# Autodesk Inventor assembly: Ellbow n24_v2
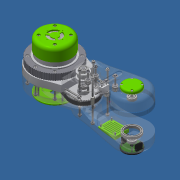
[picture p0: Inventor's stored thumbnail of the model, 180x180]
Saved by Autodesk Inventor 2016 (Build 200138000, 138)
## iProperties
Created: 2015-08-24
Part Number: Ellbow n24_v2
Material: Generisch
Document SubType Name: Assembly
Designer: 4ndreas
Mass: 4086.83 g
Surface Area: 5319.91 cm^2
Volume: 2356.13 cm^3
Density: 1.73455 g/cm^3
Author: 4ndreas
## Documents named in this file (42)
- C:\Users\4ndreas\Documents\Inventor\RobotARM v2\v4\_assemblys\Elbow.iam
- C:\Users\4ndreas\Documents\Inventor\RobotARM v2\v4\Elbow\Konstruktions-Assistent\Übertragung des Zahnriemens1.iam
- C:\Users\4ndreas\Documents\Inventor\RobotARM v2\v4\_motors\Nema24.ipt
- C:\Users\4ndreas\Documents\Inventor\RobotARM v2\v4\Elbow\Konstruktions-Assistent\Übertragung des Zahnriemens2.iam
- C:\Users\4ndreas\Documents\Inventor\RobotARM v2\v4\_printed parts\OberArm_A.ipt
- C:\Users\4ndreas\Documents\Inventor\RobotARM v2\v4\_printed parts\OberArm_B.ipt
- C:\Users\4ndreas\Documents\Inventor\RobotARM v2\v4\_misc parts\OberArm_C.ipt
- C:\Users\4ndreas\Documents\Inventor\RobotARM v2\v4\Elbow\Konstruktions-Assistent\Welle1.iam
- C:\Users\4ndreas\Documents\Inventor\Content Center Files\R2014\de-DE\DIN BEARING(1)\DIN 625 SKF - SKF 608.ipt
- C:\Users\4ndreas\Documents\Inventor\RobotARM v2\v4\_assemblys\encoder.iam
- C:\Users\4ndreas\Documents\Inventor\RobotARM v2\v4\_standard Parts\DIN 912 - M4 x 0,7 x50.ipt
- C:\Users\4ndreas\Documents\Inventor\RobotARM v2\v4\_printed parts\MotorCoverN24_3.ipt
- C:\Users\4ndreas\Documents\Inventor\RobotARM v2\v4\_printed parts\Cover_G2.ipt
- C:\Users\4ndreas\Documents\Inventor\Content Center Files\R2014\de-DE\DIN 912\DIN 912 - M3 x 0,5 x 10 x 8,75.ipt
- C:\Users\4ndreas\Documents\Inventor\Content Center Files\R2014\de-DE\DIN 912\DIN 912 - M4 x 0,7 x 35 x 20.ipt
- C:\Users\4ndreas\Documents\Inventor\Content Center Files\R2014\de-DE\DIN 912\DIN 912 - M4 x 0,7 x 40 x 20.ipt
- C:\Users\4ndreas\Documents\Inventor\Content Center Files\R2014\de-DE\DIN 9021\DIN 9021 - 4,3.ipt
- C:\Users\4ndreas\Documents\Inventor\Content Center Files\R2014\de-DE\DIN 625 - T1\DIN 625 T1 - 624 - 4 x 13 x 5.ipt
- C:\Users\4ndreas\Documents\Inventor\Content Center Files\R2014\de-DE\DIN 125-1  A\DIN 125 - A 4,3.ipt
- C:\Users\4ndreas\Documents\Inventor\Content Center Files\R2014\de-DE\DIN BEARING(1)\DIN 625 SKF - SKF 61807.ipt
- C:\Users\4ndreas\Documents\Inventor\RobotARM v2\v4\_standard Parts\DIN 912 - M4 x 0,7 x55.ipt
- C:\Users\4ndreas\Documents\Inventor\RobotARM v2\v4\_metal parts\16221600.ipt
- C:\Users\4ndreas\Documents\Inventor\Content Center Files\R2014\de-DE\DIN 912\DIN 912 - M4 x 0,7 x 30 x 20.ipt
- C:\Users\4ndreas\Documents\Inventor\Content Center Files\R2014\de-DE\DIN 933\DIN 933 - M4  x 55.ipt
- C:\Users\4ndreas\Documents\Inventor\Content Center Files\R2014\de-DE\DIN 934\DIN 934 - M4 x 0,7.ipt
- C:\Users\4ndreas\Documents\Inventor\Content Center Files\R2014\de-DE\DIN 562\DIN 562 - M4 x 7.ipt
- C:\Users\4ndreas\Documents\Inventor\Content Center Files\R2014\de-DE\DIN 933\DIN 933 - M4  x 25.ipt
- C:\Users\4ndreas\Documents\Inventor\RobotARM v2\v4\_printed parts\OberArmMagnet.ipt
- C:\Users\4ndreas\Documents\Inventor\Content Center Files\R2014\de-DE\DIN 7991(2)\DIN 7991 - M4x30.ipt
- C:\Users\4ndreas\Documents\Inventor\RobotARM v2\v4\_metal parts\Synchrone RiemenscheibeT5_z48.ipt
- C:\Users\4ndreas\Documents\Inventor\RobotARM v2\v4\_metal parts\Belt_T_Spacer.ipt
- C:\Users\4ndreas\Documents\Inventor\RobotARM v2\v4\_standard Parts\DIN 625 SKF - SKF 624_flansch.ipt
- C:\Users\4ndreas\Documents\Inventor\Content Center Files\R2014\de-DE\DIN 125-1  A\DIN 125 - A 8,4.ipt
- C:\Users\4ndreas\Documents\Inventor\Content Center Files\R2014\de-DE\DIN 933\DIN 933 - M4  x 40.ipt
- C:\Users\4ndreas\Documents\Inventor\RobotARM v2\v4\_encoder\EncoderMagnet.ipt
- C:\Users\4ndreas\Documents\Inventor\RobotARM v2\v4\_printed parts\Cable_Cover.ipt
- C:\Users\4ndreas\Documents\Inventor\RobotARM v2\v4\_metal parts\Alu_Belt_tens.ipt
- C:\Users\4ndreas\Documents\Inventor\Content Center Files\R2014\de-DE\DIN 913\DIN 913 - M4 x 16.ipt
- C:\Users\4ndreas\Documents\Inventor\RobotARM v2\v4\_standard Parts\Distanzhuelse_M4x20mm.ipt
- C:\Users\4ndreas\Documents\Inventor\Content Center Files\R2014\de-DE\DIN 913\DIN 913 - M4 x 4.ipt
- C:\Users\4ndreas\Documents\Inventor\Content Center Files\R2014\de-DE\BS EN ISO 13337\ISO 13337 - 3 x 26BS EN ISO.ipt
- C:\Users\4ndreas\Documents\Inventor\Content Center Files\R2014\de-DE\BS EN ISO 13337\ISO 13337 - 3 x 20BS EN ISO.ipt
## Components (175 placed, 40 different names)
1. Übertragung des Zahnriemens:1 [sub-assembly] — Passend:25, Passend:31, Passend:37, Passend:41, Passend:120, Passend:193
2. Nema24:1 — Passend:3, Passend:16, Winkel:1, Winkel:2, Passend:33, Passend:35, Passend:36, Passend:52, Passend:54, Passend:55, Passend:154, Passend:155, Fluchtend:11
3. Übertragung des Zahnriemens:2 [sub-assembly] — Passend:16, Passend:24, Passend:34, Passend:156
4. OberArm_A:1 — Passend:29, Fluchtend:1, Passend:30, Fluchtend:3, Passend:32, Passend:33, Passend:34, Passend:44, Passend:45, Passend:72, Passend:73, Passend:74, Passend:75, Passend:76, Passend:78, Passend:245, Passend:246, Passend:247, Passend:248, Passend:249, Passend:275, Passend:283, Winkel:3, Passend:291, Passend:292
5. OberArm_B:1 — Passend:28, Passend:29, Fluchtend:1, Passend:30, Fluchtend:4, Passend:43, Passend:50, Passend:226, Passend:227, Passend:228, Passend:229, Passend:241, Passend:242, Passend:243, Passend:244, Fluchtend:12, Passend:273
6. OberArm_C:1 — Passend:28, Fluchtend:3, Passend:31, Fluchtend:4, Passend:48, Passend:49, Passend:51, Fluchtend:9, Passend:102, Passend:103, Passend:107, Passend:108, Passend:130, Passend:131, Passend:132, Passend:133, Passend:134, Passend:135, Passend:136, Passend:137, Passend:138, Passend:144, Passend:150, Passend:151, Passend:161, Passend:162, Passend:201, Passend:202, Passend:203, Passend:204, Passend:205, Passend:211, Passend:220, Passend:222, Passend:223, Passend:250, Passend:251, Passend:252, Passend:256, Fluchtend:17, Passend:319, Passend:320, Passend:105, Passend:324, Passend:325, Passend:336, Passend:339, Passend:340
7. Cover_G2:1 — Fluchtend:9, Passend:80, Passend:81, Passend:82, Passend:83, Passend:84, Passend:85, Passend:86, Passend:87
8. Welle:1 [sub-assembly] — Passend:37, Passend:38, Passend:40, Passend:39, Passend:206, Passend:284, Passend:286, Passend:287, Tangential:1
9. encoder:1 [sub-assembly] — Passend:41, Passend:43, Passend:256
10. OberArmMagnet:1 — Fluchtend:12, Passend:261, Passend:262, Fluchtend:13, Passend:263, Passend:264, Fluchtend:14, Fluchtend:15, Passend:310, Passend:311
11. DIN 625 SKF SKF 608:1 — Passend:38, Passend:204
12. DIN 625 SKF SKF 608:2 — Passend:39, Passend:205, Passend:207
13. DIN 625 SKF SKF 608:3 — Passend:40, Passend:203
14. DIN 625 SKF SKF 608:4 — Passend:45, Passend:49
15. DIN 625 SKF SKF 608:5 — Passend:50, Passend:51
16. DIN 625 SKF SKF 608:6 — Passend:44, Passend:48
17. DIN 912 - ersetzt durch DIN EN ISO 4762 M4 x 50:5 — Passend:55, Passend:71, Passend:258
18. DIN 912 - ersetzt durch DIN EN ISO 4762 M4 x 50:6 — Passend:54, Passend:69
19. DIN 912 - ersetzt durch DIN EN ISO 4762 M4 x 50:7 — Passend:53, Passend:70
20. DIN 912 - ersetzt durch DIN EN ISO 4762 M4 x 50:8 — Passend:52, Passend:68
21. DIN 125-1 A A 4,3:6
22. DIN 125-1 A A 4,3:7
23. DIN 125-1 A A 4,3:8
24. DIN 125-1 A A 4,3:9
25. Distanzhuelse_M4x20mm:1 — Passend:71, Fluchtend:6, Fluchtend:7, Passend:72
26. Distanzhuelse_M4x20mm:2 — Passend:69, Fluchtend:6, Passend:73, Passend:88
27. Distanzhuelse_M4x20mm:3 — Passend:70, Fluchtend:7, Fluchtend:8, Passend:75, Passend:76
28. Distanzhuelse_M4x20mm:4 — Passend:68, Fluchtend:8, Passend:74, Passend:259
29. MotorCoverN24_3:1 — Passend:78, Passend:89, Passend:92, Passend:93, Passend:94, Passend:257, Passend:260
30. DIN 912 - ersetzt durch DIN EN ISO 4762 M3 x 10:1 — Passend:82, Passend:87
31. DIN 912 - ersetzt durch DIN EN ISO 4762 M3 x 10:2 — Passend:81, Passend:86
32. DIN 912 - ersetzt durch DIN EN ISO 4762 M3 x 10:3 — Passend:83, Passend:84
33. DIN 912 - ersetzt durch DIN EN ISO 4762 M3 x 10:4 — Passend:80, Passend:85
34. DIN 912 - ersetzt durch DIN EN ISO 4762 M4 x 35:1 — Passend:88, Passend:89
35. DIN 912 - ersetzt durch DIN EN ISO 4762 M4 x 35:2 — Passend:92, Passend:93, Passend:258
36. DIN 912 - ersetzt durch DIN EN ISO 4762 M4 x 35:3 — Passend:259, Passend:260
37. DIN 912 - ersetzt durch DIN EN ISO 4762 M4 x 35:4 — Passend:90, Passend:94, Passend:257
38. DIN 933 - ersetzt durch DIN EN 24017 M4  x 40:1 — Passend:96, Passend:105, Passend:109, Passend:115, Passend:121, Passend:293, Passend:296, Passend:297
39. DIN 9021 4,3:1 — Passend:96, Passend:102, Passend:298
40. DIN 9021 4,3:2 — Passend:103, Passend:303, Passend:307, Fluchtend:18
41. DIN 9021 4,3:3 — Passend:108, Passend:109, Passend:122
42. DIN 9021 4,3:4 — Passend:107, Passend:123, Passend:309, Passend:323
43. DIN 625 - T1 624 - 4 x 13 x 5:1 — Passend:110, Passend:124, Passend:294
44. F624 ZZ 4x13x5:2 — Passend:110, Passend:115, Passend:295, Passend:296
45. DIN 625 - T1 624 - 4 x 13 x 5:3 — Passend:125, Passend:304, Passend:305
46. DIN 125-1 A A 4,3:1 — Passend:117, Passend:119, Passend:125, Passend:308
47. DIN 125-1 A A 4,3:2 — Passend:117, Passend:119, Passend:120, Passend:123
48. DIN 125-1 A A 4,3:3 — Passend:116, Passend:118, Passend:124
49. DIN 125-1 A A 4,3:4 — Passend:116, Passend:118, Passend:121, Passend:122
50. DIN 625 SKF SKF 61807:1 — Passend:130, Passend:131
51. Distanzhuelse_M4x20mm:5 — Passend:132, Passend:136, Passend:137
52. Distanzhuelse_M4x20mm:6 — Passend:133, Passend:134, Passend:135
53. DIN 912 - ersetzt durch DIN EN ISO 4762 M4 x 55:12 — Passend:138
54. DIN 125-1 A A 4,3:10
55. DIN 912 - ersetzt durch DIN EN ISO 4762 M4 x 55:13 — Passend:144
56. DIN 125-1 A A 4,3:11
57. DIN 912 - ersetzt durch DIN EN ISO 4762 M4 x 55:14 — Passend:151
58. DIN 125-1 A A 4,3:12
59. DIN 912 - ersetzt durch DIN EN ISO 4762 M4 x 55:15 — Passend:150
60. DIN 125-1 A A 4,3:13
61. 16221600:1 — Passend:154, Passend:155, Fluchtend:10, Passend:345
62. Synchrone RiemenscheibeT5_z48:1 — Passend:156, Fluchtend:10, Passend:285, Passend:289, Passend:341, Passend:342
63. DIN 912 - ersetzt durch DIN EN ISO 4762 M4 x 55:16 — Passend:162, Passend:190
64. DIN 912 - ersetzt durch DIN EN ISO 4762 M4 x 55:17 — Passend:161, Passend:165, Passend:188
65. DIN 125-1 A A 4,3:14
66. DIN 125-1 A A 4,3:15
67. DIN 912 - ersetzt durch DIN EN ISO 4762 M4 x 30:1 — Passend:165, Passend:187
68. DIN 125-1 A A 4,3:16
69. DIN 125-1 A A 4,3:17
70. DIN 933 - ersetzt durch DIN EN 24017 M4  x 55:2 — Passend:184, Passend:191, Passend:192, Passend:198
71. DIN 933 - ersetzt durch DIN EN 24017 M4  x 55:1 — Passend:183, Passend:194, Passend:196
72. DIN 125-1 A A 4,3:18
73. DIN 125-1 A A 4,3:19
74. DIN 934 - ersetzt durch DIN EN 24032/28673/28674 M4:1 — Passend:188
75. DIN 934 - ersetzt durch DIN EN 24032/28673/28674 M4:2 — Passend:187
76. DIN 934 - ersetzt durch DIN EN 24032/28673/28674 M4:3 — Passend:184
77. DIN 934 - ersetzt durch DIN EN 24032/28673/28674 M4:4 — Passend:183
78. DIN 934 - ersetzt durch DIN EN 24032/28673/28674 M4:6 — Passend:190
79. DIN 625 - T1 624 - 4 x 13 x 5:5 — Passend:193, Passend:195, Passend:197
80. DIN 625 - T1 624 - 4 x 13 x 5:6 — Passend:192, Passend:199, Passend:201
81. DIN 625 - T1 624 - 4 x 13 x 5:7 — Passend:191, Passend:199, Passend:200
82. DIN 625 - T1 624 - 4 x 13 x 5:8 — Passend:194, Passend:195, Passend:202
83. DIN 934 - ersetzt durch DIN EN 24032/28673/28674 M4:7 — Passend:196, Passend:197
84. DIN 934 - ersetzt durch DIN EN 24032/28673/28674 M4:8 — Passend:198, Passend:200
85. 16221600:2 — Passend:206, Passend:207, Passend:288, Passend:343, Passend:344
86. DIN 912 - ersetzt durch DIN EN ISO 4762 M4 x 55:18 — Passend:211, Passend:239
87. DIN 125-1 A A 4,3:20
88. DIN 912 - ersetzt durch DIN EN ISO 4762 M4 x 55:19 — Passend:220, Passend:240
89. DIN 912 - ersetzt durch DIN EN ISO 4762 M4 x 55:20 — Passend:222, Passend:238
90. DIN 912 - ersetzt durch DIN EN ISO 4762 M4 x 55:21 — Passend:223, Passend:237
91. DIN 125-1 A A 4,3:21
92. DIN 125-1 A A 4,3:5
93. DIN 125-1 A A 4,3:22
94. DIN 562 M4:1 — Passend:239, Passend:245, Passend:246
95. DIN 562 M4:2 — Passend:240, Passend:241, Passend:242
96. DIN 562 M4:3 — Passend:237, Passend:247, Passend:248
97. DIN 562 M4:4 — Passend:238, Passend:243, Passend:244
98. DIN 933 - ersetzt durch DIN EN 24017 M4  x 25:1 — Passend:250, Passend:251, Passend:252, Passend:254
99. DIN 934 - ersetzt durch DIN EN 24032/28673/28674 M4:9 — Passend:254
100. DIN 7991 M4x30:2 — Passend:262, Fluchtend:13, Passend:267
101. DIN 7991 M4x30:3 — Passend:263, Fluchtend:14, Passend:266
102. DIN 7991 M4x30:4 — Passend:264, Fluchtend:15, Passend:269
103. DIN 7991 M4x30:1 — Passend:268
104. DIN 934 - ersetzt durch DIN EN 24032/28673/28674 M4:10 — Passend:268, Passend:272
105. DIN 934 - ersetzt durch DIN EN 24032/28673/28674 M4:11 — Passend:267, Passend:271, Passend:272, Passend:273
106. DIN 934 - ersetzt durch DIN EN 24032/28673/28674 M4:12 — Passend:269, Passend:270
107. DIN 934 - ersetzt durch DIN EN 24032/28673/28674 M4:13 — Passend:266, Passend:270, Passend:271
108. Belt_T_Spacer:1 — Passend:274, Passend:275, Passend:281, Winkel:3
109. DIN 912 - ersetzt durch DIN EN ISO 4762 M4 x 40:11 — Passend:274, Passend:276, Passend:277, Passend:278, Passend:282, Passend:283, Passend:290
110. F624 ZZ 4x13x5:1 — Passend:276, Passend:280, Passend:281
111. DIN 625 - T1 624 - 4 x 13 x 5:9 — Passend:278, Passend:279, Passend:282
112. DIN 125-1 A A 4,3:37 — Passend:277, Passend:279, Passend:280
113. DIN 125-1 A A 8,4:1 — Passend:284, Passend:285
114. DIN 125-1 A A 8,4:2 — Passend:287, Passend:288
115. DIN 125-1 A A 8,4:3 — Passend:286, Passend:289
116. DIN 562 M4:5 — Passend:290, Passend:291, Passend:292
117. DIN 125-1 A A 4,3:38 — Passend:293, Passend:294, Passend:295
118. DIN 934 - ersetzt durch DIN EN 24032/28673/28674 M4:14 — Passend:297, Passend:298
119. F624 ZZ 4x13x5:3 — Passend:299, Passend:300, Passend:302
120. DIN 933 - ersetzt durch DIN EN 24017 M4  x 40:2 — Passend:299, Passend:300, Passend:301, Passend:303, Passend:305, Passend:306, Passend:308, Passend:309, Passend:322
121. DIN 934 - ersetzt durch DIN EN 24032/28673/28674 M4:15 — Passend:306, Passend:307
122. DIN 125-1 A A 4,3:39 — Passend:301, Passend:302, Passend:304
123. EncoderMagnet:1 — Passend:310, Passend:311
124. Cable_Cover:1 — Fluchtend:17, Passend:312, Passend:313, Passend:314, Passend:315, Passend:316, Passend:317, Passend:318, Passend:321
125. DIN 912 - ersetzt durch DIN EN ISO 4762 M3 x 10:5 — Passend:314, Passend:316
126. DIN 912 - ersetzt durch DIN EN ISO 4762 M3 x 10:6 — Passend:315, Passend:319, Passend:321
127. DIN 912 - ersetzt durch DIN EN ISO 4762 M3 x 10:7 — Passend:313, Passend:317
128. DIN 912 - ersetzt durch DIN EN ISO 4762 M3 x 10:8 — Passend:312, Passend:318, Passend:320
129. Alu_Belt_tens:1 — Passend:322, Passend:323, Passend:328, Passend:332, Passend:338
130. DIN 912 - ersetzt durch DIN EN ISO 4762 M4 x 30:18 — Passend:328, Passend:329, Passend:330, Passend:331, Passend:333, Passend:335
131. DIN 9021 4,3:5 — Passend:329, Fluchtend:18, Passend:330
132. DIN 9021 4,3:7 — Passend:331, Passend:332, Passend:334
133. DIN 934 - ersetzt durch DIN EN 24032/28673/28674 M4:16 — Passend:333, Passend:334
134. DIN 934 - ersetzt durch DIN EN 24032/28673/28674 M4:17 — Passend:336, Passend:337, Passend:339, Passend:340
135. DIN 913 M4 x 16:1 — Passend:337, Passend:338
136. DIN 913 M4 x 4:1 — Passend:341, Tangential:1
137. BS EN ISO 13337 3 x 26:1 — Passend:342
138. DIN 913 M4 x 4:2 — Passend:343
139. BS EN ISO 13337 3 x 20:1 — Passend:344
140. DIN 913 M4 x 4:3 — Passend:345
141. DIN 912 - ersetzt durch DIN EN ISO 4762 M4 x 30:5 — Passend:229
142. DIN 125-1 A A 4,3:23
143. Distanzhuelse_M4x20mm:7 — Passend:226, Passend:227, Passend:228, Passend:235
144. DIN 912 - ersetzt durch DIN EN ISO 4762 M4 x 30:4 — Passend:235
145. DIN 125-1 A A 4,3:24
146. DIN 912 - ersetzt durch DIN EN ISO 4762 M4 x 30:6
147. DIN 125-1 A A 4,3:25
148. Distanzhuelse_M4x20mm:8
149. DIN 912 - ersetzt durch DIN EN ISO 4762 M4 x 30:7
150. DIN 125-1 A A 4,3:26
151. DIN 912 - ersetzt durch DIN EN ISO 4762 M4 x 30:8
152. DIN 125-1 A A 4,3:27
153. Distanzhuelse_M4x20mm:9
154. DIN 912 - ersetzt durch DIN EN ISO 4762 M4 x 30:9
155. DIN 125-1 A A 4,3:28
156. DIN 912 - ersetzt durch DIN EN ISO 4762 M4 x 30:10
157. DIN 125-1 A A 4,3:29
158. Distanzhuelse_M4x20mm:10
159. DIN 912 - ersetzt durch DIN EN ISO 4762 M4 x 30:11
160. DIN 125-1 A A 4,3:30
161. DIN 912 - ersetzt durch DIN EN ISO 4762 M4 x 30:12
162. DIN 125-1 A A 4,3:31
163. Distanzhuelse_M4x20mm:11
164. DIN 912 - ersetzt durch DIN EN ISO 4762 M4 x 30:13
165. DIN 125-1 A A 4,3:32
166. DIN 912 - ersetzt durch DIN EN ISO 4762 M4 x 30:14
167. DIN 125-1 A A 4,3:33
168. Distanzhuelse_M4x20mm:12
169. DIN 912 - ersetzt durch DIN EN ISO 4762 M4 x 30:15
170. DIN 125-1 A A 4,3:34
171. DIN 912 - ersetzt durch DIN EN ISO 4762 M4 x 30:16
172. DIN 125-1 A A 4,3:35
173. Distanzhuelse_M4x20mm:13
174. DIN 912 - ersetzt durch DIN EN ISO 4762 M4 x 30:17
175. DIN 125-1 A A 4,3:36
## Component patterns: (7 elements, first: DIN 912 - ersetzt durch DIN EN ISO 4762 M4 x 30:5 + DIN 125-1 A A 4,3:23 + Distanzhuelse_M4x20mm:7 + DIN 912 - ersetzt durch DIN EN ISO 4762 M4 x 30:4 + DIN 125-1 A A 4,3:24)
## Relationships (316: Mate 296, Flush 16, Angle 3, Tangent 1)
- Passend:3 [Mate]: Nema24:1
- Passend:12 [Mate]
- Passend:13 [Mate]
- Passend:16 [Mate]: Nema24:1 ↔ Übertragung des Zahnriemens:2
- Winkel:1 [Angle] (0 deg): Nema24:1
- Passend:24 [Mate]: Übertragung des Zahnriemens:2
- Passend:25 [Mate]: Übertragung des Zahnriemens:1
- Winkel:2 [Angle] (180 deg): Nema24:1
- Passend:28 [Mate]: OberArm_B:1 ↔ OberArm_C:1
- Passend:29 [Mate]: OberArm_A:1 ↔ OberArm_B:1
- Fluchtend:1 [Flush]: OberArm_A:1 ↔ OberArm_B:1
- Passend:30 [Mate]: OberArm_A:1 ↔ OberArm_B:1
- Fluchtend:3 [Flush]: OberArm_A:1 ↔ OberArm_C:1
- Passend:31 [Mate]: Übertragung des Zahnriemens:1 ↔ OberArm_C:1
- Passend:32 [Mate]: OberArm_A:1
- Passend:33 [Mate]: Nema24:1 ↔ OberArm_A:1
- Passend:34 [Mate]: Übertragung des Zahnriemens:2 ↔ OberArm_A:1
- Passend:35 [Mate]: Nema24:1
- Passend:36 [Mate]: Nema24:1
- Fluchtend:4 [Flush]: OberArm_B:1 ↔ OberArm_C:1
- Passend:37 [Mate]: Übertragung des Zahnriemens:1 ↔ Welle:1
- Passend:38 [Mate]: Welle:1 ↔ DIN 625 SKF SKF 608:1
- Passend:39 [Mate]: Welle:1 ↔ DIN 625 SKF SKF 608:2
- Passend:40 [Mate]: Welle:1 ↔ DIN 625 SKF SKF 608:3
- Passend:41 [Mate]: Übertragung des Zahnriemens:1 ↔ encoder:1
- Passend:43 [Mate]: OberArm_B:1 ↔ encoder:1
- Passend:44 [Mate]: OberArm_A:1 ↔ DIN 625 SKF SKF 608:6
- Passend:45 [Mate]: OberArm_A:1 ↔ DIN 625 SKF SKF 608:4
- Passend:48 [Mate]: OberArm_C:1 ↔ DIN 625 SKF SKF 608:6
- Passend:49 [Mate]: OberArm_C:1 ↔ DIN 625 SKF SKF 608:4
- Passend:50 [Mate]: OberArm_B:1 ↔ DIN 625 SKF SKF 608:5
- Passend:51 [Mate]: OberArm_C:1 ↔ DIN 625 SKF SKF 608:5
- Passend:52 [Mate]: Nema24:1 ↔ DIN 912 - ersetzt durch DIN EN ISO 4762 M4 x 50:8
- Passend:53 [Mate]: DIN 912 - ersetzt durch DIN EN ISO 4762 M4 x 50:7
- Passend:54 [Mate]: Nema24:1 ↔ DIN 912 - ersetzt durch DIN EN ISO 4762 M4 x 50:6
- Passend:55 [Mate]: Nema24:1 ↔ DIN 912 - ersetzt durch DIN EN ISO 4762 M4 x 50:5
- [Mate]: DIN 912 - ersetzt durch DIN EN ISO 4762 M4 x 50:8 ↔ DIN 125-1 A A 4,3:7
- [Mate]: DIN 912 - ersetzt durch DIN EN ISO 4762 M4 x 50:6 ↔ DIN 125-1 A A 4,3:6
- [Mate]: DIN 912 - ersetzt durch DIN EN ISO 4762 M4 x 50:5 ↔ DIN 125-1 A A 4,3:9
- [Mate]: DIN 912 - ersetzt durch DIN EN ISO 4762 M4 x 50:7 ↔ DIN 125-1 A A 4,3:8
- [Mate]: DIN 912 - ersetzt durch DIN EN ISO 4762 M4 x 50:7 ↔ DIN 125-1 A A 4,3:8
- [Mate]: DIN 912 - ersetzt durch DIN EN ISO 4762 M4 x 50:8 ↔ DIN 125-1 A A 4,3:7
- [Mate]: DIN 912 - ersetzt durch DIN EN ISO 4762 M4 x 50:6 ↔ DIN 125-1 A A 4,3:6
- [Mate]: DIN 912 - ersetzt durch DIN EN ISO 4762 M4 x 50:5 ↔ DIN 125-1 A A 4,3:9
- [Mate]: Nema24:1 ↔ DIN 125-1 A A 4,3:6
- [Mate]: Nema24:1 ↔ DIN 125-1 A A 4,3:7
- [Mate]: Nema24:1 ↔ DIN 125-1 A A 4,3:9
- [Mate]: Nema24:1 ↔ DIN 125-1 A A 4,3:8
- Passend:68 [Mate]: DIN 912 - ersetzt durch DIN EN ISO 4762 M4 x 50:8 ↔ Distanzhuelse_M4x20mm:4
- Passend:69 [Mate]: DIN 912 - ersetzt durch DIN EN ISO 4762 M4 x 50:6 ↔ Distanzhuelse_M4x20mm:2
- Passend:70 [Mate]: DIN 912 - ersetzt durch DIN EN ISO 4762 M4 x 50:7 ↔ Distanzhuelse_M4x20mm:3
- Passend:71 [Mate]: DIN 912 - ersetzt durch DIN EN ISO 4762 M4 x 50:5 ↔ Distanzhuelse_M4x20mm:1
- Fluchtend:6 [Flush]: Distanzhuelse_M4x20mm:1 ↔ Distanzhuelse_M4x20mm:2
- Fluchtend:7 [Flush]: Distanzhuelse_M4x20mm:1 ↔ Distanzhuelse_M4x20mm:3
- Fluchtend:8 [Flush]: Distanzhuelse_M4x20mm:3 ↔ Distanzhuelse_M4x20mm:4
- Passend:72 [Mate]: OberArm_A:1 ↔ Distanzhuelse_M4x20mm:1
- Passend:73 [Mate]: OberArm_A:1 ↔ Distanzhuelse_M4x20mm:2
- Passend:74 [Mate]: OberArm_A:1 ↔ Distanzhuelse_M4x20mm:4
- Passend:75 [Mate]: OberArm_A:1 ↔ Distanzhuelse_M4x20mm:3
- Passend:76 [Mate]: OberArm_A:1 ↔ Distanzhuelse_M4x20mm:3
- Passend:78 [Mate]: OberArm_A:1 ↔ MotorCoverN24_3:1
- Fluchtend:9 [Flush]: OberArm_C:1 ↔ Cover_G2:1
- Passend:80 [Mate]: Cover_G2:1 ↔ DIN 912 - ersetzt durch DIN EN ISO 4762 M3 x 10:4
- Passend:81 [Mate]: Cover_G2:1 ↔ DIN 912 - ersetzt durch DIN EN ISO 4762 M3 x 10:2
- Passend:82 [Mate]: Cover_G2:1 ↔ DIN 912 - ersetzt durch DIN EN ISO 4762 M3 x 10:1
- Passend:83 [Mate]: Cover_G2:1 ↔ DIN 912 - ersetzt durch DIN EN ISO 4762 M3 x 10:3
- Passend:84 [Mate]: Cover_G2:1 ↔ DIN 912 - ersetzt durch DIN EN ISO 4762 M3 x 10:3
- Passend:85 [Mate]: Cover_G2:1 ↔ DIN 912 - ersetzt durch DIN EN ISO 4762 M3 x 10:4
- Passend:86 [Mate]: Cover_G2:1 ↔ DIN 912 - ersetzt durch DIN EN ISO 4762 M3 x 10:2
- Passend:87 [Mate]: Cover_G2:1 ↔ DIN 912 - ersetzt durch DIN EN ISO 4762 M3 x 10:1
- Passend:88 [Mate]: Distanzhuelse_M4x20mm:2 ↔ DIN 912 - ersetzt durch DIN EN ISO 4762 M4 x 35:1
- Passend:89 [Mate]: MotorCoverN24_3:1 ↔ DIN 912 - ersetzt durch DIN EN ISO 4762 M4 x 35:1
- Passend:90 [Mate]: DIN 912 - ersetzt durch DIN EN ISO 4762 M4 x 35:4
- Passend:92 [Mate]: MotorCoverN24_3:1 ↔ DIN 912 - ersetzt durch DIN EN ISO 4762 M4 x 35:2
- Passend:93 [Mate]: MotorCoverN24_3:1 ↔ DIN 912 - ersetzt durch DIN EN ISO 4762 M4 x 35:2
- Passend:94 [Mate]: MotorCoverN24_3:1 ↔ DIN 912 - ersetzt durch DIN EN ISO 4762 M4 x 35:4
- Passend:96 [Mate]: DIN 933 - ersetzt durch DIN EN 24017 M4  x 40:1 ↔ DIN 9021 4,3:1
- Passend:102 [Mate]: OberArm_C:1 ↔ DIN 9021 4,3:1
- Passend:103 [Mate]: OberArm_C:1 ↔ DIN 9021 4,3:2
- Passend:105 [Mate]: OberArm_C:1 ↔ DIN 933 - ersetzt durch DIN EN 24017 M4  x 40:1
- Passend:107 [Mate]: OberArm_C:1 ↔ DIN 9021 4,3:4
- Passend:108 [Mate]: OberArm_C:1 ↔ DIN 9021 4,3:3
- Passend:109 [Mate]: DIN 933 - ersetzt durch DIN EN 24017 M4  x 40:1 ↔ DIN 9021 4,3:3
- Passend:110 [Mate]: DIN 625 - T1 624 - 4 x 13 x 5:1 ↔ F624 ZZ 4x13x5:2
- Passend:115 [Mate]: DIN 933 - ersetzt durch DIN EN 24017 M4  x 40:1 ↔ F624 ZZ 4x13x5:2
- Passend:116 [Mate]: DIN 125-1 A A 4,3:3 ↔ DIN 125-1 A A 4,3:4
- Passend:117 [Mate]: DIN 125-1 A A 4,3:1 ↔ DIN 125-1 A A 4,3:2
- Passend:118 [Mate]: DIN 125-1 A A 4,3:3 ↔ DIN 125-1 A A 4,3:4
- Passend:119 [Mate]: DIN 125-1 A A 4,3:1 ↔ DIN 125-1 A A 4,3:2
- Passend:120 [Mate]: Übertragung des Zahnriemens:1 ↔ DIN 125-1 A A 4,3:2
- Passend:121 [Mate]: DIN 933 - ersetzt durch DIN EN 24017 M4  x 40:1 ↔ DIN 125-1 A A 4,3:4
- Passend:122 [Mate]: DIN 9021 4,3:3 ↔ DIN 125-1 A A 4,3:4
- Passend:123 [Mate]: DIN 9021 4,3:4 ↔ DIN 125-1 A A 4,3:2
- Passend:124 [Mate]: DIN 625 - T1 624 - 4 x 13 x 5:1 ↔ DIN 125-1 A A 4,3:3
- Passend:125 [Mate]: DIN 625 - T1 624 - 4 x 13 x 5:3 ↔ DIN 125-1 A A 4,3:1
- Passend:130 [Mate]: OberArm_C:1 ↔ DIN 625 SKF SKF 61807:1
- Passend:131 [Mate]: OberArm_C:1 ↔ DIN 625 SKF SKF 61807:1
- Passend:132 [Mate]: OberArm_C:1 ↔ Distanzhuelse_M4x20mm:5
- Passend:133 [Mate]: OberArm_C:1 ↔ Distanzhuelse_M4x20mm:6
- Passend:134 [Mate]: OberArm_C:1 ↔ Distanzhuelse_M4x20mm:6
- Passend:135 [Mate]: OberArm_C:1 ↔ Distanzhuelse_M4x20mm:6
- Passend:136 [Mate]: OberArm_C:1 ↔ Distanzhuelse_M4x20mm:5
- Passend:137 [Mate]: OberArm_C:1 ↔ Distanzhuelse_M4x20mm:5
- Passend:138 [Mate]: OberArm_C:1 ↔ DIN 912 - ersetzt durch DIN EN ISO 4762 M4 x 55:12
- [Mate]: DIN 912 - ersetzt durch DIN EN ISO 4762 M4 x 55:12 ↔ DIN 125-1 A A 4,3:10
- [Mate]: DIN 912 - ersetzt durch DIN EN ISO 4762 M4 x 55:12 ↔ DIN 125-1 A A 4,3:10
- [Mate]: OberArm_C:1 ↔ DIN 125-1 A A 4,3:10
- [Mate]: DIN 912 - ersetzt durch DIN EN ISO 4762 M4 x 55:13 ↔ DIN 125-1 A A 4,3:11
- [Mate]: DIN 912 - ersetzt durch DIN EN ISO 4762 M4 x 55:13 ↔ DIN 125-1 A A 4,3:11
- Passend:144 [Mate]: OberArm_C:1 ↔ DIN 912 - ersetzt durch DIN EN ISO 4762 M4 x 55:13
- [Mate]: OberArm_C:1 ↔ DIN 125-1 A A 4,3:11
- [Mate]: DIN 912 - ersetzt durch DIN EN ISO 4762 M4 x 55:14 ↔ DIN 125-1 A A 4,3:12
- [Mate]: DIN 912 - ersetzt durch DIN EN ISO 4762 M4 x 55:14 ↔ DIN 125-1 A A 4,3:12
- [Mate]: DIN 912 - ersetzt durch DIN EN ISO 4762 M4 x 55:15 ↔ DIN 125-1 A A 4,3:13
- [Mate]: DIN 912 - ersetzt durch DIN EN ISO 4762 M4 x 55:15 ↔ DIN 125-1 A A 4,3:13
- Passend:150 [Mate]: OberArm_C:1 ↔ DIN 912 - ersetzt durch DIN EN ISO 4762 M4 x 55:15
- Passend:151 [Mate]: OberArm_C:1 ↔ DIN 912 - ersetzt durch DIN EN ISO 4762 M4 x 55:14
- [Mate]: OberArm_C:1 ↔ DIN 125-1 A A 4,3:12
- [Mate]: OberArm_C:1 ↔ DIN 125-1 A A 4,3:13
- Passend:154 [Mate]: Nema24:1 ↔ 16221600:1
- Passend:155 [Mate] (1 mm): Nema24:1 ↔ 16221600:1
- Passend:156 [Mate]: Übertragung des Zahnriemens:2 ↔ Synchrone RiemenscheibeT5_z48:1
- Fluchtend:10 [Flush]: 16221600:1 ↔ Synchrone RiemenscheibeT5_z48:1
- Fluchtend:11 [Flush] (7 mm): Nema24:1
- [Mate]: DIN 912 - ersetzt durch DIN EN ISO 4762 M4 x 55:17 ↔ DIN 125-1 A A 4,3:15
- [Mate]: DIN 912 - ersetzt durch DIN EN ISO 4762 M4 x 55:16 ↔ DIN 125-1 A A 4,3:14
- [Mate]: DIN 912 - ersetzt durch DIN EN ISO 4762 M4 x 55:16 ↔ DIN 125-1 A A 4,3:14
- [Mate]: DIN 912 - ersetzt durch DIN EN ISO 4762 M4 x 55:17 ↔ DIN 125-1 A A 4,3:15
- Passend:161 [Mate]: OberArm_C:1 ↔ DIN 912 - ersetzt durch DIN EN ISO 4762 M4 x 55:17
- Passend:162 [Mate]: OberArm_C:1 ↔ DIN 912 - ersetzt durch DIN EN ISO 4762 M4 x 55:16
- [Mate]: OberArm_C:1 ↔ DIN 125-1 A A 4,3:14
- [Mate]: OberArm_C:1 ↔ DIN 125-1 A A 4,3:15
- Passend:165 [Mate]: DIN 912 - ersetzt durch DIN EN ISO 4762 M4 x 55:17 ↔ DIN 912 - ersetzt durch DIN EN ISO 4762 M4 x 30:1
- [Mate]: DIN 912 - ersetzt durch DIN EN ISO 4762 M4 x 30:1 ↔ DIN 125-1 A A 4,3:17
- [Mate]: DIN 912 - ersetzt durch DIN EN ISO 4762 M4 x 30:1 ↔ DIN 125-1 A A 4,3:17
- [Mate]: OberArm_C:1 ↔ DIN 125-1 A A 4,3:16
- [Mate]: OberArm_C:1 ↔ DIN 125-1 A A 4,3:17
- [Mate]: Übertragung des Zahnriemens:1 ↔ DIN 933 - ersetzt durch DIN EN 24017 M4  x 55:2
- [Mate]: Übertragung des Zahnriemens:1 ↔ DIN 933 - ersetzt durch DIN EN 24017 M4  x 55:1
- [Mate]: OberArm_C:1 ↔ DIN 933 - ersetzt durch DIN EN 24017 M4  x 55:2
- [Mate]: OberArm_C:1 ↔ DIN 933 - ersetzt durch DIN EN 24017 M4  x 55:1
- [Mate]: OberArm_C:1 ↔ DIN 933 - ersetzt durch DIN EN 24017 M4  x 55:2
- [Mate]: OberArm_C:1 ↔ DIN 933 - ersetzt durch DIN EN 24017 M4  x 55:1
- [Mate]: OberArm_C:1 ↔ DIN 125-1 A A 4,3:18
- [Mate]: OberArm_C:1 ↔ DIN 125-1 A A 4,3:19
- [Mate]: DIN 933 - ersetzt durch DIN EN 24017 M4  x 55:2 ↔ DIN 125-1 A A 4,3:19
- [Mate]: DIN 933 - ersetzt durch DIN EN 24017 M4  x 55:1 ↔ DIN 125-1 A A 4,3:18
- Passend:183 [Mate]: DIN 933 - ersetzt durch DIN EN 24017 M4  x 55:1 ↔ DIN 934 - ersetzt durch DIN EN 24032/28673/28674 M4:4
- Passend:184 [Mate]: DIN 933 - ersetzt durch DIN EN 24017 M4  x 55:2 ↔ DIN 934 - ersetzt durch DIN EN 24032/28673/28674 M4:3
- [Mate]: DIN 125-1 A A 4,3:19 ↔ DIN 934 - ersetzt durch DIN EN 24032/28673/28674 M4:3
- [Mate]: DIN 125-1 A A 4,3:18 ↔ DIN 934 - ersetzt durch DIN EN 24032/28673/28674 M4:4
- Passend:187 [Mate]: DIN 912 - ersetzt durch DIN EN ISO 4762 M4 x 30:1 ↔ DIN 934 - ersetzt durch DIN EN 24032/28673/28674 M4:2
- Passend:188 [Mate]: DIN 912 - ersetzt durch DIN EN ISO 4762 M4 x 55:17 ↔ DIN 934 - ersetzt durch DIN EN 24032/28673/28674 M4:1
- Passend:190 [Mate]: DIN 912 - ersetzt durch DIN EN ISO 4762 M4 x 55:16 ↔ DIN 934 - ersetzt durch DIN EN 24032/28673/28674 M4:6
- Passend:191 [Mate]: DIN 933 - ersetzt durch DIN EN 24017 M4  x 55:2 ↔ DIN 625 - T1 624 - 4 x 13 x 5:7
- Passend:192 [Mate]: DIN 933 - ersetzt durch DIN EN 24017 M4  x 55:2 ↔ DIN 625 - T1 624 - 4 x 13 x 5:6
- Passend:193 [Mate]: Übertragung des Zahnriemens:1 ↔ DIN 625 - T1 624 - 4 x 13 x 5:5
- Passend:194 [Mate]: DIN 933 - ersetzt durch DIN EN 24017 M4  x 55:1 ↔ DIN 625 - T1 624 - 4 x 13 x 5:8
- Passend:195 [Mate]: DIN 625 - T1 624 - 4 x 13 x 5:5 ↔ DIN 625 - T1 624 - 4 x 13 x 5:8
- Passend:196 [Mate]: DIN 933 - ersetzt durch DIN EN 24017 M4  x 55:1 ↔ DIN 934 - ersetzt durch DIN EN 24032/28673/28674 M4:7
- Passend:197 [Mate]: DIN 625 - T1 624 - 4 x 13 x 5:5 ↔ DIN 934 - ersetzt durch DIN EN 24032/28673/28674 M4:7
- Passend:198 [Mate]: DIN 933 - ersetzt durch DIN EN 24017 M4  x 55:2 ↔ DIN 934 - ersetzt durch DIN EN 24032/28673/28674 M4:8
- Passend:199 [Mate]: DIN 625 - T1 624 - 4 x 13 x 5:6 ↔ DIN 625 - T1 624 - 4 x 13 x 5:7
- Passend:200 [Mate]: DIN 625 - T1 624 - 4 x 13 x 5:7 ↔ DIN 934 - ersetzt durch DIN EN 24032/28673/28674 M4:8
- Passend:201 [Mate]: OberArm_C:1 ↔ DIN 625 - T1 624 - 4 x 13 x 5:6
- Passend:202 [Mate]: OberArm_C:1 ↔ DIN 625 - T1 624 - 4 x 13 x 5:8
- Passend:203 [Mate]: OberArm_C:1 ↔ DIN 625 SKF SKF 608:3
- Passend:204 [Mate]: OberArm_C:1 ↔ DIN 625 SKF SKF 608:1
- Passend:205 [Mate]: OberArm_C:1 ↔ DIN 625 SKF SKF 608:2
- Passend:206 [Mate]: Welle:1 ↔ 16221600:2
- Passend:207 [Mate] (0.5 mm): DIN 625 SKF SKF 608:2 ↔ 16221600:2
- [Mate]: DIN 912 - ersetzt durch DIN EN ISO 4762 M4 x 55:18 ↔ DIN 125-1 A A 4,3:20
- [Mate]: DIN 912 - ersetzt durch DIN EN ISO 4762 M4 x 55:18 ↔ DIN 125-1 A A 4,3:20
- [Mate]: OberArm_C:1 ↔ DIN 125-1 A A 4,3:20
- Passend:211 [Mate]: OberArm_C:1 ↔ DIN 912 - ersetzt durch DIN EN ISO 4762 M4 x 55:18
- [Mate]: DIN 912 - ersetzt durch DIN EN ISO 4762 M4 x 55:19 ↔ DIN 125-1 A A 4,3:21
- [Mate]: DIN 912 - ersetzt durch DIN EN ISO 4762 M4 x 55:20 ↔ DIN 125-1 A A 4,3:22
- [Mate]: DIN 912 - ersetzt durch DIN EN ISO 4762 M4 x 55:21 ↔ DIN 125-1 A A 4,3:5
- [Mate]: DIN 912 - ersetzt durch DIN EN ISO 4762 M4 x 55:20 ↔ DIN 125-1 A A 4,3:22
- [Mate]: DIN 912 - ersetzt durch DIN EN ISO 4762 M4 x 55:19 ↔ DIN 125-1 A A 4,3:21
- [Mate]: DIN 912 - ersetzt durch DIN EN ISO 4762 M4 x 55:21 ↔ DIN 125-1 A A 4,3:5
- Passend:220 [Mate]: OberArm_C:1 ↔ DIN 912 - ersetzt durch DIN EN ISO 4762 M4 x 55:19
- [Mate]: OberArm_C:1 ↔ DIN 125-1 A A 4,3:21
- Passend:222 [Mate]: OberArm_C:1 ↔ DIN 912 - ersetzt durch DIN EN ISO 4762 M4 x 55:20
- Passend:223 [Mate]: OberArm_C:1 ↔ DIN 912 - ersetzt durch DIN EN ISO 4762 M4 x 55:21
- [Mate]: OberArm_C:1 ↔ DIN 125-1 A A 4,3:5
- [Mate]: OberArm_C:1 ↔ DIN 125-1 A A 4,3:22
- Passend:226 [Mate]: OberArm_B:1 ↔ Distanzhuelse_M4x20mm:7
- Passend:227 [Mate]: OberArm_B:1 ↔ Distanzhuelse_M4x20mm:7
- Passend:228 [Mate]: OberArm_B:1 ↔ Distanzhuelse_M4x20mm:7
- Passend:229 [Mate]: OberArm_B:1 ↔ DIN 912 - ersetzt durch DIN EN ISO 4762 M4 x 30:5
- [Mate]: DIN 912 - ersetzt durch DIN EN ISO 4762 M4 x 30:5 ↔ DIN 125-1 A A 4,3:23
- [Mate]: DIN 912 - ersetzt durch DIN EN ISO 4762 M4 x 30:5 ↔ DIN 125-1 A A 4,3:23
- [Mate]: OberArm_B:1 ↔ DIN 125-1 A A 4,3:23
- [Mate]: DIN 912 - ersetzt durch DIN EN ISO 4762 M4 x 30:4 ↔ DIN 125-1 A A 4,3:24
- [Mate]: DIN 912 - ersetzt durch DIN EN ISO 4762 M4 x 30:4 ↔ DIN 125-1 A A 4,3:24
- Passend:235 [Mate]: Distanzhuelse_M4x20mm:7 ↔ DIN 912 - ersetzt durch DIN EN ISO 4762 M4 x 30:4
- [Mate]: OberArm_A:1 ↔ DIN 125-1 A A 4,3:24
- Passend:237 [Mate]: DIN 912 - ersetzt durch DIN EN ISO 4762 M4 x 55:21 ↔ DIN 562 M4:3
- Passend:238 [Mate]: DIN 912 - ersetzt durch DIN EN ISO 4762 M4 x 55:20 ↔ DIN 562 M4:4
- Passend:239 [Mate]: DIN 912 - ersetzt durch DIN EN ISO 4762 M4 x 55:18 ↔ DIN 562 M4:1
- Passend:240 [Mate]: DIN 912 - ersetzt durch DIN EN ISO 4762 M4 x 55:19 ↔ DIN 562 M4:2
- Passend:241 [Mate]: OberArm_B:1 ↔ DIN 562 M4:2
- Passend:242 [Mate]: OberArm_B:1 ↔ DIN 562 M4:2
- Passend:243 [Mate]: OberArm_B:1 ↔ DIN 562 M4:4
- Passend:244 [Mate]: OberArm_B:1 ↔ DIN 562 M4:4
- Passend:245 [Mate]: OberArm_A:1 ↔ DIN 562 M4:1
- Passend:246 [Mate]: OberArm_A:1 ↔ DIN 562 M4:1
- Passend:247 [Mate]: OberArm_A:1 ↔ DIN 562 M4:3
- Passend:248 [Mate]: OberArm_A:1 ↔ DIN 562 M4:3
- Passend:249 [Mate]: OberArm_A:1
- Passend:250 [Mate]: OberArm_C:1 ↔ DIN 933 - ersetzt durch DIN EN 24017 M4  x 25:1
- Passend:251 [Mate]: OberArm_C:1 ↔ DIN 933 - ersetzt durch DIN EN 24017 M4  x 25:1
- Passend:252 [Mate]: OberArm_C:1 ↔ DIN 933 - ersetzt durch DIN EN 24017 M4  x 25:1
- [Mate]: DIN 125-1 A A 4,3:16 ↔ DIN 933 - ersetzt durch DIN EN 24017 M4  x 25:1
- Passend:254 [Mate]: DIN 933 - ersetzt durch DIN EN 24017 M4  x 25:1 ↔ DIN 934 - ersetzt durch DIN EN 24032/28673/28674 M4:9
- [Mate]: DIN 125-1 A A 4,3:16 ↔ DIN 934 - ersetzt durch DIN EN 24032/28673/28674 M4:9
- Passend:256 [Mate]: OberArm_C:1 ↔ encoder:1
- Passend:257 [Mate]: MotorCoverN24_3:1 ↔ DIN 912 - ersetzt durch DIN EN ISO 4762 M4 x 35:4
- Passend:258 [Mate]: DIN 912 - ersetzt durch DIN EN ISO 4762 M4 x 50:5 ↔ DIN 912 - ersetzt durch DIN EN ISO 4762 M4 x 35:2
- Passend:259 [Mate]: Distanzhuelse_M4x20mm:4 ↔ DIN 912 - ersetzt durch DIN EN ISO 4762 M4 x 35:3
- Passend:260 [Mate]: MotorCoverN24_3:1 ↔ DIN 912 - ersetzt durch DIN EN ISO 4762 M4 x 35:3
- Fluchtend:12 [Flush]: OberArm_B:1 ↔ OberArmMagnet:1
- Passend:261 [Mate]: OberArmMagnet:1
- Passend:262 [Mate]: OberArmMagnet:1 ↔ DIN 7991 M4x30:2
- Fluchtend:13 [Flush]: OberArmMagnet:1 ↔ DIN 7991 M4x30:2
- Passend:263 [Mate]: OberArmMagnet:1 ↔ DIN 7991 M4x30:3
- Passend:264 [Mate]: OberArmMagnet:1 ↔ DIN 7991 M4x30:4
- Fluchtend:14 [Flush]: OberArmMagnet:1 ↔ DIN 7991 M4x30:3
- Fluchtend:15 [Flush]: OberArmMagnet:1 ↔ DIN 7991 M4x30:4
- [Mate]: OberArmMagnet:1 ↔ DIN 7991 M4x30:1
- [Flush]: OberArmMagnet:1 ↔ DIN 7991 M4x30:1
- Passend:266 [Mate]: DIN 7991 M4x30:3 ↔ DIN 934 - ersetzt durch DIN EN 24032/28673/28674 M4:13
- Passend:267 [Mate]: DIN 7991 M4x30:2 ↔ DIN 934 - ersetzt durch DIN EN 24032/28673/28674 M4:11
- Passend:268 [Mate]: DIN 7991 M4x30:1 ↔ DIN 934 - ersetzt durch DIN EN 24032/28673/28674 M4:10
- Passend:269 [Mate]: DIN 7991 M4x30:4 ↔ DIN 934 - ersetzt durch DIN EN 24032/28673/28674 M4:12
- Passend:270 [Mate]: DIN 934 - ersetzt durch DIN EN 24032/28673/28674 M4:12 ↔ DIN 934 - ersetzt durch DIN EN 24032/28673/28674 M4:13
- Passend:271 [Mate]: DIN 934 - ersetzt durch DIN EN 24032/28673/28674 M4:11 ↔ DIN 934 - ersetzt durch DIN EN 24032/28673/28674 M4:13
- Passend:272 [Mate]: DIN 934 - ersetzt durch DIN EN 24032/28673/28674 M4:10 ↔ DIN 934 - ersetzt durch DIN EN 24032/28673/28674 M4:11
- Passend:273 [Mate]: OberArm_B:1 ↔ DIN 934 - ersetzt durch DIN EN 24032/28673/28674 M4:11
- Passend:274 [Mate]: Belt_T_Spacer:1 ↔ DIN 912 - ersetzt durch DIN EN ISO 4762 M4 x 40:11
- Passend:275 [Mate]: OberArm_A:1 ↔ Belt_T_Spacer:1
- Passend:276 [Mate]: DIN 912 - ersetzt durch DIN EN ISO 4762 M4 x 40:11 ↔ F624 ZZ 4x13x5:1
- Passend:277 [Mate]: DIN 912 - ersetzt durch DIN EN ISO 4762 M4 x 40:11 ↔ DIN 125-1 A A 4,3:37
- Passend:278 [Mate]: DIN 912 - ersetzt durch DIN EN ISO 4762 M4 x 40:11 ↔ DIN 625 - T1 624 - 4 x 13 x 5:9
- Passend:279 [Mate]: DIN 625 - T1 624 - 4 x 13 x 5:9 ↔ DIN 125-1 A A 4,3:37
- Passend:280 [Mate]: F624 ZZ 4x13x5:1 ↔ DIN 125-1 A A 4,3:37
- Passend:281 [Mate]: Belt_T_Spacer:1 ↔ F624 ZZ 4x13x5:1
- Passend:282 [Mate]: DIN 912 - ersetzt durch DIN EN ISO 4762 M4 x 40:11 ↔ DIN 625 - T1 624 - 4 x 13 x 5:9
- Passend:283 [Mate]: OberArm_A:1 ↔ DIN 912 - ersetzt durch DIN EN ISO 4762 M4 x 40:11
- Winkel:3 [Angle] (180 deg): OberArm_A:1 ↔ Belt_T_Spacer:1
- Passend:284 [Mate]: Welle:1 ↔ DIN 125-1 A A 8,4:1
- Passend:285 [Mate]: Synchrone RiemenscheibeT5_z48:1 ↔ DIN 125-1 A A 8,4:1
- Passend:286 [Mate]: Welle:1 ↔ DIN 125-1 A A 8,4:3
- Passend:287 [Mate]: Welle:1 ↔ DIN 125-1 A A 8,4:2
- Passend:288 [Mate]: 16221600:2 ↔ DIN 125-1 A A 8,4:2
- Passend:289 [Mate]: Synchrone RiemenscheibeT5_z48:1 ↔ DIN 125-1 A A 8,4:3
- Passend:290 [Mate]: DIN 912 - ersetzt durch DIN EN ISO 4762 M4 x 40:11 ↔ DIN 562 M4:5
- Passend:291 [Mate]: OberArm_A:1 ↔ DIN 562 M4:5
- Passend:292 [Mate]: OberArm_A:1 ↔ DIN 562 M4:5
- Passend:293 [Mate]: DIN 933 - ersetzt durch DIN EN 24017 M4  x 40:1 ↔ DIN 125-1 A A 4,3:38
- Passend:294 [Mate]: DIN 625 - T1 624 - 4 x 13 x 5:1 ↔ DIN 125-1 A A 4,3:38
- Passend:295 [Mate]: F624 ZZ 4x13x5:2 ↔ DIN 125-1 A A 4,3:38
- Passend:296 [Mate]: DIN 933 - ersetzt durch DIN EN 24017 M4  x 40:1 ↔ F624 ZZ 4x13x5:2
- Passend:297 [Mate]: DIN 933 - ersetzt durch DIN EN 24017 M4  x 40:1 ↔ DIN 934 - ersetzt durch DIN EN 24032/28673/28674 M4:14
- Passend:298 [Mate]: DIN 9021 4,3:1 ↔ DIN 934 - ersetzt durch DIN EN 24032/28673/28674 M4:14
- Passend:299 [Mate]: F624 ZZ 4x13x5:3 ↔ DIN 933 - ersetzt durch DIN EN 24017 M4  x 40:2
- Passend:300 [Mate]: F624 ZZ 4x13x5:3 ↔ DIN 933 - ersetzt durch DIN EN 24017 M4  x 40:2
- Passend:301 [Mate]: DIN 933 - ersetzt durch DIN EN 24017 M4  x 40:2 ↔ DIN 125-1 A A 4,3:39
- Passend:302 [Mate]: F624 ZZ 4x13x5:3 ↔ DIN 125-1 A A 4,3:39
- Passend:303 [Mate]: DIN 9021 4,3:2 ↔ DIN 933 - ersetzt durch DIN EN 24017 M4  x 40:2
- Passend:304 [Mate]: DIN 625 - T1 624 - 4 x 13 x 5:3 ↔ DIN 125-1 A A 4,3:39
- Passend:305 [Mate]: DIN 625 - T1 624 - 4 x 13 x 5:3 ↔ DIN 933 - ersetzt durch DIN EN 24017 M4  x 40:2
- Passend:306 [Mate]: DIN 933 - ersetzt durch DIN EN 24017 M4  x 40:2 ↔ DIN 934 - ersetzt durch DIN EN 24032/28673/28674 M4:15
- Passend:307 [Mate]: DIN 9021 4,3:2 ↔ DIN 934 - ersetzt durch DIN EN 24032/28673/28674 M4:15
- Passend:308 [Mate]: DIN 125-1 A A 4,3:1 ↔ DIN 933 - ersetzt durch DIN EN 24017 M4  x 40:2
- Passend:309 [Mate]: DIN 9021 4,3:4 ↔ DIN 933 - ersetzt durch DIN EN 24017 M4  x 40:2
- Passend:310 [Mate]: OberArmMagnet:1 ↔ EncoderMagnet:1
- Passend:311 [Mate]: OberArmMagnet:1 ↔ EncoderMagnet:1
- Fluchtend:17 [Flush]: OberArm_C:1 ↔ Cable_Cover:1
- Passend:312 [Mate]: Cable_Cover:1 ↔ DIN 912 - ersetzt durch DIN EN ISO 4762 M3 x 10:8
- Passend:313 [Mate]: Cable_Cover:1 ↔ DIN 912 - ersetzt durch DIN EN ISO 4762 M3 x 10:7
- Passend:314 [Mate]: Cable_Cover:1 ↔ DIN 912 - ersetzt durch DIN EN ISO 4762 M3 x 10:5
- Passend:315 [Mate]: Cable_Cover:1 ↔ DIN 912 - ersetzt durch DIN EN ISO 4762 M3 x 10:6
- Passend:316 [Mate]: Cable_Cover:1 ↔ DIN 912 - ersetzt durch DIN EN ISO 4762 M3 x 10:5
- Passend:317 [Mate]: Cable_Cover:1 ↔ DIN 912 - ersetzt durch DIN EN ISO 4762 M3 x 10:7
- Passend:318 [Mate]: Cable_Cover:1 ↔ DIN 912 - ersetzt durch DIN EN ISO 4762 M3 x 10:8
- Passend:319 [Mate]: OberArm_C:1 ↔ DIN 912 - ersetzt durch DIN EN ISO 4762 M3 x 10:6
- Passend:320 [Mate]: OberArm_C:1 ↔ DIN 912 - ersetzt durch DIN EN ISO 4762 M3 x 10:8
- Passend:321 [Mate]: Cable_Cover:1 ↔ DIN 912 - ersetzt durch DIN EN ISO 4762 M3 x 10:6
- Passend:322 [Mate]: DIN 933 - ersetzt durch DIN EN 24017 M4  x 40:2 ↔ Alu_Belt_tens:1
- Passend:323 [Mate]: DIN 9021 4,3:4 ↔ Alu_Belt_tens:1
- Passend:324 [Mate]: OberArm_C:1
- Passend:325 [Mate]: OberArm_C:1
- Passend:326 [Mate]
- Passend:327 [Mate]
- Passend:328 [Mate]: Alu_Belt_tens:1 ↔ DIN 912 - ersetzt durch DIN EN ISO 4762 M4 x 30:18
- Passend:329 [Mate]: DIN 912 - ersetzt durch DIN EN ISO 4762 M4 x 30:18 ↔ DIN 9021 4,3:5
- Fluchtend:18 [Flush]: DIN 9021 4,3:2 ↔ DIN 9021 4,3:5
- Passend:330 [Mate]: DIN 912 - ersetzt durch DIN EN ISO 4762 M4 x 30:18 ↔ DIN 9021 4,3:5
- Passend:331 [Mate]: DIN 912 - ersetzt durch DIN EN ISO 4762 M4 x 30:18 ↔ DIN 9021 4,3:7
- Passend:332 [Mate]: Alu_Belt_tens:1 ↔ DIN 9021 4,3:7
- Passend:333 [Mate]: DIN 912 - ersetzt durch DIN EN ISO 4762 M4 x 30:18 ↔ DIN 934 - ersetzt durch DIN EN 24032/28673/28674 M4:16
- Passend:334 [Mate]: DIN 9021 4,3:7 ↔ DIN 934 - ersetzt durch DIN EN 24032/28673/28674 M4:16
- Passend:335 [Mate]: DIN 912 - ersetzt durch DIN EN ISO 4762 M4 x 30:18
- Passend:336 [Mate]: OberArm_C:1 ↔ DIN 934 - ersetzt durch DIN EN 24032/28673/28674 M4:17
- Passend:337 [Mate]: DIN 934 - ersetzt durch DIN EN 24032/28673/28674 M4:17 ↔ DIN 913 M4 x 16:1
- Passend:338 [Mate]: Alu_Belt_tens:1 ↔ DIN 913 M4 x 16:1
- Passend:339 [Mate]: OberArm_C:1 ↔ DIN 934 - ersetzt durch DIN EN 24032/28673/28674 M4:17
- Passend:340 [Mate]: OberArm_C:1 ↔ DIN 934 - ersetzt durch DIN EN 24032/28673/28674 M4:17
- Passend:341 [Mate]: Synchrone RiemenscheibeT5_z48:1 ↔ DIN 913 M4 x 4:1
- Tangential:1: Welle:1 ↔ DIN 913 M4 x 4:1
- Passend:342 [Mate]: Synchrone RiemenscheibeT5_z48:1 ↔ BS EN ISO 13337 3 x 26:1
- Passend:343 [Mate]: 16221600:2 ↔ DIN 913 M4 x 4:2
- Passend:344 [Mate]: 16221600:2 ↔ BS EN ISO 13337 3 x 20:1
- Passend:345 [Mate]: 16221600:1 ↔ DIN 913 M4 x 4:3
